# Autodesk Inventor assembly: Tiny_House_Trailer
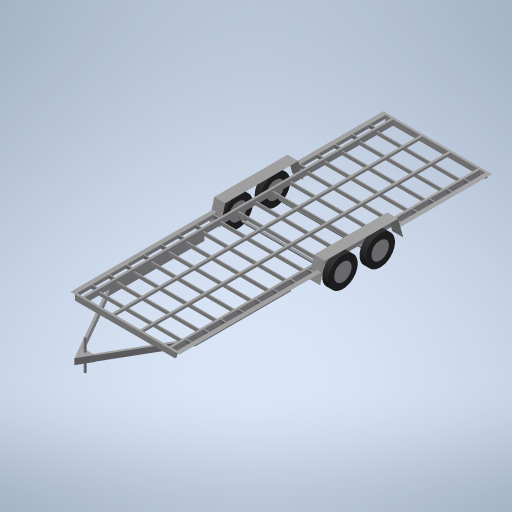
[picture p0: Inventor's stored thumbnail of the model, 512x512]
Saved by Autodesk Inventor 2024 (Build 280153000, 153)
## iProperties
Created: 2017-07-15
Part Number: Tiny_House_Trailer
Document SubType Name: Assembly
Designer: thoma
Author: thoma
## Documents named in this file (19)
- C:\Users\Tom\Documents\Tom_Levers_Public_Git_Repository\Inventor\Tiny-House_Trailer\Tiny_House_Trailer.iam
- C:\Users\Tom\Documents\Tom_Levers_Public_Git_Repository\Inventor\Tiny-House_Trailer\Beam--Sides.ipt
- C:\Users\Tom\Documents\Tom_Levers_Public_Git_Repository\Inventor\Tiny-House_Trailer\Beam--Front_and_Back.ipt
- C:\Users\Tom\Documents\Tom_Levers_Public_Git_Repository\Inventor\Tiny-House_Trailer\Outrigger.ipt
- C:\Users\Tom\Documents\Tom_Levers_Public_Git_Repository\Inventor\Tiny-House_Trailer\Outrigger_MIR.ipt
- C:\Users\Tom\Documents\Tom_Levers_Public_Git_Repository\Inventor\Tiny-House_Trailer\Angle--Anterior--Right.ipt
- C:\Users\Tom\Documents\Tom_Levers_Public_Git_Repository\Inventor\Tiny-House_Trailer\Angle--Posterior--Right.ipt
- C:\Users\Tom\Documents\Tom_Levers_Public_Git_Repository\Inventor\Tiny-House_Trailer\Angle--Anterior--Left.ipt
- C:\Users\Tom\Documents\Tom_Levers_Public_Git_Repository\Inventor\Tiny-House_Trailer\Angle--Posterior--Left.ipt
- C:\Users\Tom\Documents\Tom_Levers_Public_Git_Repository\Inventor\Tiny-House_Trailer\Fender.ipt
- C:\Users\Tom\Documents\Tom_Levers_Public_Git_Repository\Inventor\Tiny-House_Trailer\Fender_MIR.ipt
- C:\Users\Tom\Documents\Tom_Levers_Public_Git_Repository\Inventor\Tiny-House_Trailer\Beam--2x2.ipt
- C:\Users\Tom\Documents\Tom_Levers_Public_Git_Repository\Inventor\Tiny-House_Trailer\Beam--1x3.ipt
- C:\Users\Tom\Documents\Tom_Levers_Public_Git_Repository\Inventor\Tiny-House_Trailer\Wheel_and_Tire.iam
- C:\Users\Tom\Documents\Tom_Levers_Public_Git_Repository\Inventor\Tiny-House_Trailer\Wheel_and_Tire_MIR.iam
- C:\Users\Tom\Documents\Tom_Levers_Public_Git_Repository\Inventor\Tiny-House_Trailer\Wheel_and_Tire_MIR1.iam
- C:\Users\Tom\Documents\Tom_Levers_Public_Git_Repository\Inventor\Tiny-House_Trailer\Wheel_and_Tire_MIR_MIR.iam
- C:\Users\Tom\Documents\Tom_Levers_Public_Git_Repository\Inventor\Tiny-House_Trailer\Hauling_Wishbone.ipt
- C:\Users\Tom\Documents\Tom_Levers_Public_Git_Repository\Inventor\Tiny-House_Trailer\Drop_Axle.ipt
## Components (62 placed, 18 different names)
1. Beam--Sides:1 — Flush:1, Mate:1, Flush:2, Flush:5, Mate:3, Flush:6, Flush:7, Mate:4, Flush:9, Mate:5, Flush:11, Mate:6, Flush:13, Mate:7, Flush:15, Mate:8, Flush:17, Mate:9, Flush:19, Mate:10, Flush:21, Mate:11, Flush:31, Mate:16, Flush:33, Mate:17, Flush:35, Mate:18, Flush:37, Mate:19, Flush:39, Mate:20, Flush:41, Flush:43, Mate:25, Flush:49, Mate:29, Flush:90
2. Beam--Front_and_Back:1 — Flush:1, Mate:1, Flush:2, Mate:2, Flush:3, Flush:4, Flush:8, Flush:10, Flush:12, Flush:14, Flush:16, Flush:18, Flush:20, Flush:22, Flush:32, Flush:34, Flush:36, Flush:38, Flush:40, Mate:21, Flush:42, Flush:45, Mate:23, Flush:46, Mate:28, Flush:50, Mate:30, Flush:51, Flush:88, Flush:89
3. Beam--Sides:2 — Mate:2, Flush:3, Flush:4, Mate:27, Mate:31, Mate:32, Mate:33, Mate:34, Mate:35, Mate:36, Mate:37, Mate:38, Mate:39, Mate:40, Mate:41, Mate:42, Mate:43, Mate:44, Mate:45, Mate:46, Mate:47
4. Beam--Front_and_Back:2 — Flush:5, Mate:3, Flush:6, Mate:22, Flush:44, Flush:47, Mate:24, Flush:48, Mate:26
5. Outrigger:1 — Flush:7, Mate:4, Flush:8
6. Outrigger:2 — Flush:9, Mate:5, Flush:10
7. Outrigger:3 — Flush:11, Mate:6, Flush:12
8. Outrigger:4 — Flush:13, Mate:7, Flush:14
9. Outrigger:5 — Flush:15, Mate:8, Flush:16
10. Outrigger:6 — Flush:17, Mate:9, Flush:18
11. Outrigger:7 — Flush:19, Mate:10, Flush:20
12. Outrigger:8 — Flush:21, Mate:11, Flush:22
13. Outrigger:13 — Flush:31, Mate:16, Flush:32
14. Outrigger:14 — Flush:33, Mate:17, Flush:34
15. Outrigger:15 — Flush:35, Mate:18, Flush:36
16. Outrigger:16 — Flush:37, Mate:19, Flush:38
17. Outrigger:17 — Flush:39, Mate:20, Flush:40
18. Outrigger_MIR:1 — Flush:53
19. Outrigger_MIR:2 — Flush:55
20. Outrigger_MIR:3 — Flush:57
21. Outrigger_MIR:4 — Flush:59
22. Outrigger_MIR:5 — Flush:61
23. Outrigger_MIR:6 — Flush:63
24. Outrigger_MIR:7 — Flush:65
25. Outrigger_MIR:8 — Flush:67
26. Outrigger_MIR:13
27. Outrigger_MIR:14
28. Outrigger_MIR:15
29. Outrigger_MIR:16
30. Outrigger_MIR:17
31. Angle--Anterior--Right:1 — Flush:41, Mate:21, Flush:42
32. Angle--Posterior--Right:1 — Flush:43, Mate:22, Flush:44
33. Angle--Anterior--Left:1 — Flush:45, Mate:23, Flush:46
34. Angle--Posterior--Left:1 — Flush:47, Mate:24, Flush:48
35. Fender:1 — Mate:25, Flush:49, Mate:26, Flush:86, Flush:87, Mate:48
36. Fender_MIR:1
37. Beam--2x2:1 — Mate:29, Mate:30, Flush:51
38. Beam--2x2:2 — Mate:27, Mate:28, Flush:50, Flush:52, Flush:54, Flush:56, Flush:58, Flush:60, Flush:62, Flush:64, Flush:66, Flush:68, Flush:70, Flush:72, Flush:74, Flush:76, Flush:78, Flush:80, Flush:82, Flush:84
39. Beam--1x3:1 — Mate:31, Flush:52, Flush:53
40. Beam--1x3:2 — Mate:32, Flush:54, Flush:55
41. Beam--1x3:3 — Mate:33, Flush:56, Flush:57
42. Beam--1x3:4 — Mate:34, Flush:58, Flush:59
43. Beam--1x3:5 — Mate:35, Flush:60, Flush:61
44. Beam--1x3:6 — Mate:36, Flush:62, Flush:63
45. Beam--1x3:7 — Mate:37, Flush:64, Flush:65
46. Beam--1x3:8 — Mate:38, Flush:66, Flush:67, Flush:69
47. Beam--1x3:9 — Mate:39, Flush:68, Flush:69, Flush:71
48. Beam--1x3:10 — Mate:40, Flush:70, Flush:71, Flush:73
49. Beam--1x3:11 — Mate:41, Flush:72, Flush:73, Flush:75
50. Beam--1x3:12 — Mate:42, Flush:74, Flush:75, Flush:77
51. Beam--1x3:13 — Mate:43, Flush:76, Flush:77, Flush:79
52. Beam--1x3:14 — Mate:44, Flush:78, Flush:79, Flush:81
53. Beam--1x3:15 — Mate:45, Flush:80, Flush:81, Flush:83
54. Beam--1x3:16 — Mate:46, Flush:82, Flush:83, Flush:85
55. Beam--1x3:17 — Mate:47, Flush:84, Flush:85
56. Wheel_and_Tire:1 [sub-assembly] — Flush:86, Flush:87, Mate:48, Mate:49, Mate:50, Mate:51, Mate:52
57. Wheel_and_Tire_MIR:1 [sub-assembly]
58. Wheel_and_Tire_MIR1:1 [sub-assembly]
59. Wheel_and_Tire_MIR_MIR:1 [sub-assembly]
60. Hauling_Wishbone:1 — Flush:88, Flush:89, Flush:90
61. Drop_Axle:1 — Mate:49, Mate:50, Mate:51, Flush:91, Flush:92
62. Drop_Axle:2 — Flush:91, Mate:52, Flush:92
## Relationships (132: Flush 84, Mate 48)
- Flush:1: Beam--Sides:1 ↔ Beam--Front_and_Back:1
- Mate:1: Beam--Sides:1 ↔ Beam--Front_and_Back:1
- Flush:2 (-127 mm): Beam--Sides:1 ↔ Beam--Front_and_Back:1
- Mate:2: Beam--Front_and_Back:1 ↔ Beam--Sides:2
- Flush:3: Beam--Front_and_Back:1 ↔ Beam--Sides:2
- Flush:4 (127 mm): Beam--Front_and_Back:1 ↔ Beam--Sides:2
- Flush:5: Beam--Sides:1 ↔ Beam--Front_and_Back:2
- Mate:3: Beam--Sides:1 ↔ Beam--Front_and_Back:2
- Flush:6 (-127 mm): Beam--Sides:1 ↔ Beam--Front_and_Back:2
- Flush:7: Beam--Sides:1 ↔ Outrigger:1
- Mate:4: Beam--Sides:1 ↔ Outrigger:1
- Flush:8 (381 mm): Beam--Front_and_Back:1 ↔ Outrigger:1
- Flush:9: Beam--Sides:1 ↔ Outrigger:2
- Mate:5: Beam--Sides:1 ↔ Outrigger:2
- Flush:10 (787.4 mm): Beam--Front_and_Back:1 ↔ Outrigger:2
- Flush:11: Beam--Sides:1 ↔ Outrigger:3
- Mate:6: Beam--Sides:1 ↔ Outrigger:3
- Flush:12 (1193.8 mm): Beam--Front_and_Back:1 ↔ Outrigger:3
- Flush:13: Beam--Sides:1 ↔ Outrigger:4
- Mate:7: Beam--Sides:1 ↔ Outrigger:4
- Flush:14 (1600.2 mm): Beam--Front_and_Back:1 ↔ Outrigger:4
- Flush:15: Beam--Sides:1 ↔ Outrigger:5
- Mate:8: Beam--Sides:1 ↔ Outrigger:5
- Flush:16 (2006.6 mm): Beam--Front_and_Back:1 ↔ Outrigger:5
- Flush:17: Beam--Sides:1 ↔ Outrigger:6
- Mate:9: Beam--Sides:1 ↔ Outrigger:6
- Flush:18 (2413 mm): Beam--Front_and_Back:1 ↔ Outrigger:6
- Flush:19: Beam--Sides:1 ↔ Outrigger:7
- Mate:10: Beam--Sides:1 ↔ Outrigger:7
- Flush:20 (2819.4 mm): Beam--Front_and_Back:1 ↔ Outrigger:7
- Flush:21: Beam--Sides:1 ↔ Outrigger:8
- Mate:11: Beam--Sides:1 ↔ Outrigger:8
- Flush:22 (3225.8 mm): Beam--Front_and_Back:1 ↔ Outrigger:8
- Flush:31: Beam--Sides:1 ↔ Outrigger:13
- Mate:16: Beam--Sides:1 ↔ Outrigger:13
- Flush:32 (5257.8 mm): Beam--Front_and_Back:1 ↔ Outrigger:13
- Flush:33: Beam--Sides:1 ↔ Outrigger:14
- Mate:17: Beam--Sides:1 ↔ Outrigger:14
- Flush:34 (5664.2 mm): Beam--Front_and_Back:1 ↔ Outrigger:14
- Flush:35: Beam--Sides:1 ↔ Outrigger:15
- Mate:18: Beam--Sides:1 ↔ Outrigger:15
- Flush:36 (6070.6 mm): Beam--Front_and_Back:1 ↔ Outrigger:15
- Flush:37: Beam--Sides:1 ↔ Outrigger:16
- Mate:19: Beam--Sides:1 ↔ Outrigger:16
- Flush:38 (6477 mm): Beam--Front_and_Back:1 ↔ Outrigger:16
- Flush:39: Beam--Sides:1 ↔ Outrigger:17
- Mate:20: Beam--Sides:1 ↔ Outrigger:17
- Flush:40 (6883.4 mm): Beam--Front_and_Back:1 ↔ Outrigger:17
- Flush:41: Beam--Sides:1 ↔ Angle--Anterior--Right:1
- Mate:21: Beam--Front_and_Back:1 ↔ Angle--Anterior--Right:1
- Flush:42: Beam--Front_and_Back:1 ↔ Angle--Anterior--Right:1
- Flush:43: Beam--Sides:1 ↔ Angle--Posterior--Right:1
- Mate:22: Beam--Front_and_Back:2 ↔ Angle--Posterior--Right:1
- Flush:44: Beam--Front_and_Back:2 ↔ Angle--Posterior--Right:1
- Flush:45: Beam--Front_and_Back:1 ↔ Angle--Anterior--Left:1
- Mate:23: Beam--Front_and_Back:1 ↔ Angle--Anterior--Left:1
- Flush:46: Beam--Front_and_Back:1 ↔ Angle--Anterior--Left:1
- Flush:47: Beam--Front_and_Back:2 ↔ Angle--Posterior--Left:1
- Mate:24: Beam--Front_and_Back:2 ↔ Angle--Posterior--Left:1
- Flush:48: Beam--Front_and_Back:2 ↔ Angle--Posterior--Left:1
- Mate:25: Beam--Sides:1 ↔ Fender:1
- Flush:49 (-215.9 mm): Beam--Sides:1 ↔ Fender:1
- Mate:26 (-3073.4 mm): Beam--Front_and_Back:2 ↔ Fender:1
- Mate:27 (660.4 mm): Beam--Sides:2 ↔ Beam--2x2:2
- Mate:28: Beam--Front_and_Back:1 ↔ Beam--2x2:2
- Flush:50: Beam--Front_and_Back:1 ↔ Beam--2x2:2
- Mate:29 (660.4 mm): Beam--Sides:1 ↔ Beam--2x2:1
- Mate:30: Beam--Front_and_Back:1 ↔ Beam--2x2:1
- Flush:51: Beam--Front_and_Back:1 ↔ Beam--2x2:1
- Mate:31: Beam--Sides:2 ↔ Beam--1x3:1
- Flush:52 (50.8 mm): Beam--2x2:2 ↔ Beam--1x3:1
- Flush:53: Outrigger_MIR:1 ↔ Beam--1x3:1
- Mate:32: Beam--Sides:2 ↔ Beam--1x3:2
- Flush:54 (50.8 mm): Beam--2x2:2 ↔ Beam--1x3:2
- Flush:55: Outrigger_MIR:2 ↔ Beam--1x3:2
- Mate:33: Beam--Sides:2 ↔ Beam--1x3:3
- Flush:56 (50.8 mm): Beam--2x2:2 ↔ Beam--1x3:3
- Flush:57: Outrigger_MIR:3 ↔ Beam--1x3:3
- Mate:34: Beam--Sides:2 ↔ Beam--1x3:4
- Flush:58 (50.8 mm): Beam--2x2:2 ↔ Beam--1x3:4
- Flush:59: Outrigger_MIR:4 ↔ Beam--1x3:4
- Mate:35: Beam--Sides:2 ↔ Beam--1x3:5
- Flush:60 (50.8 mm): Beam--2x2:2 ↔ Beam--1x3:5
- Flush:61: Outrigger_MIR:5 ↔ Beam--1x3:5
- Mate:36: Beam--Sides:2 ↔ Beam--1x3:6
- Flush:62 (50.8 mm): Beam--2x2:2 ↔ Beam--1x3:6
- Flush:63: Outrigger_MIR:6 ↔ Beam--1x3:6
- Mate:37: Beam--Sides:2 ↔ Beam--1x3:7
- Flush:64 (50.8 mm): Beam--2x2:2 ↔ Beam--1x3:7
- Flush:65: Outrigger_MIR:7 ↔ Beam--1x3:7
- Mate:38: Beam--Sides:2 ↔ Beam--1x3:8
- Flush:66 (50.8 mm): Beam--2x2:2 ↔ Beam--1x3:8
- Flush:67: Outrigger_MIR:8 ↔ Beam--1x3:8
- Mate:39: Beam--Sides:2 ↔ Beam--1x3:9
- Flush:68 (50.8 mm): Beam--2x2:2 ↔ Beam--1x3:9
- Flush:69 (406.4 mm): Beam--1x3:8 ↔ Beam--1x3:9
- Mate:40: Beam--Sides:2 ↔ Beam--1x3:10
- Flush:70 (50.8 mm): Beam--2x2:2 ↔ Beam--1x3:10
- Flush:71 (406.4 mm): Beam--1x3:9 ↔ Beam--1x3:10
- Mate:41: Beam--Sides:2 ↔ Beam--1x3:11
- Flush:72 (50.8 mm): Beam--2x2:2 ↔ Beam--1x3:11
- Flush:73 (406.4 mm): Beam--1x3:10 ↔ Beam--1x3:11
- Mate:42: Beam--Sides:2 ↔ Beam--1x3:12
- Flush:74 (50.8 mm): Beam--2x2:2 ↔ Beam--1x3:12
- Flush:75 (406.4 mm): Beam--1x3:11 ↔ Beam--1x3:12
- Mate:43: Beam--Sides:2 ↔ Beam--1x3:13
- Flush:76 (50.8 mm): Beam--2x2:2 ↔ Beam--1x3:13
- Flush:77 (406.4 mm): Beam--1x3:12 ↔ Beam--1x3:13
- Mate:44: Beam--Sides:2 ↔ Beam--1x3:14
- Flush:78 (50.8 mm): Beam--2x2:2 ↔ Beam--1x3:14
- Flush:79 (406.4 mm): Beam--1x3:13 ↔ Beam--1x3:14
- Mate:45: Beam--Sides:2 ↔ Beam--1x3:15
- Flush:80 (50.8 mm): Beam--2x2:2 ↔ Beam--1x3:15
- Flush:81 (406.4 mm): Beam--1x3:14 ↔ Beam--1x3:15
- Mate:46: Beam--Sides:2 ↔ Beam--1x3:16
- Flush:82 (50.8 mm): Beam--2x2:2 ↔ Beam--1x3:16
- Flush:83 (406.4 mm): Beam--1x3:15 ↔ Beam--1x3:16
- Mate:47: Beam--Sides:2 ↔ Beam--1x3:17
- Flush:84 (50.8 mm): Beam--2x2:2 ↔ Beam--1x3:17
- Flush:85 (406.4 mm): Beam--1x3:16 ↔ Beam--1x3:17
- Flush:86: Fender:1 ↔ Wheel_and_Tire:1
- Flush:87: Fender:1 ↔ Wheel_and_Tire:1
- Mate:48 (534.2128 mm): Fender:1 ↔ Wheel_and_Tire:1
- Flush:88: Beam--Front_and_Back:1 ↔ Hauling_Wishbone:1
- Flush:89 (127 mm): Beam--Front_and_Back:1 ↔ Hauling_Wishbone:1
- Flush:90: Beam--Sides:1 ↔ Hauling_Wishbone:1
- Mate:49: Wheel_and_Tire:1 ↔ Drop_Axle:1
- Mate:50: Wheel_and_Tire:1 ↔ Drop_Axle:1
- Mate:51: Wheel_and_Tire:1 ↔ Drop_Axle:1
- Flush:91 (-878.7638 mm): Drop_Axle:1 ↔ Drop_Axle:2
- Mate:52: Wheel_and_Tire:1 ↔ Drop_Axle:2
- Flush:92: Drop_Axle:1 ↔ Drop_Axle:2
